# Autodesk Inventor assembly: Z Belt Drive Unit B
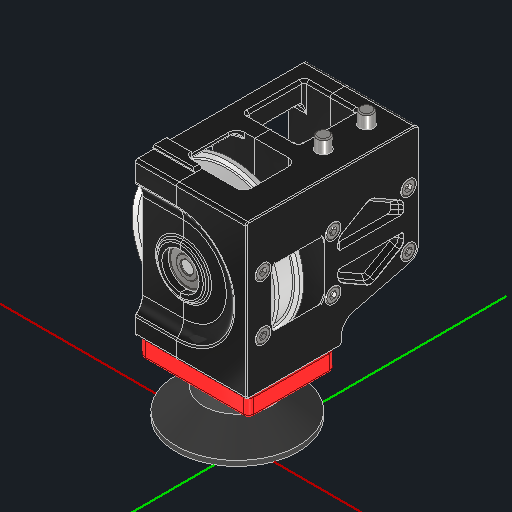
[picture p0: Inventor's stored thumbnail of the model, 512x512]
Saved by Autodesk Inventor 2022.2 (Build 262287010, 287A)
## iProperties
Created: 2022-03-12
Part Number: Z Belt Drive Unit B
Document SubType Name: Assembly
Designer: sleib
Author: sleib
## Documents named in this file (11)
- C:\Users\sleib\Projekte\Voron-2\CAD\Inventor\Z Belt-Drive Unit [B].iam
- C:\Users\sleib\Projekte\Voron-2\CAD\Inventor\Z Belt-Drive Body [B].ipt
- C:\Users\sleib\Projekte\Voron-2\CAD\Inventor\M3 Threaded Insert.ipt
- C:\Users\sleib\Projekte\Voron-2\CAD\Inventor\M3x40 SHCS.ipt
- C:\Users\sleib\Projekte\Voron-2\CAD\Inventor\M5x40 SHCS.ipt
- C:\Users\sleib\Projekte\Voron-2\CAD\Inventor\Z Belt-Drive Shaft.iam
- C:\Users\sleib\Projekte\Voron-2\CAD\Inventor\Z Belt-Drive Base-Plate [B].ipt
- C:\Users\sleib\Projekte\Voron-2\CAD\Inventor\M5x10 BHCS.ipt
- C:\Users\sleib\Projekte\Voron-2\CAD\Inventor\M5 Hexnut.ipt
- C:\Users\sleib\Projekte\Voron-2\CAD\Inventor\Rubber Compressor Foot.ipt
- C:\Users\sleib\Projekte\Voron-2\CAD\Inventor\M3x8 SHCS.ipt
## Components (26 placed, 10 different names)
1. Z Belt-Drive Body [B]:1 — Passend:1, Passend:2, Passend:3, Passend:4, Passend:5, Passend:6, Fluchtend:1, Fluchtend:2, Fluchtend:3, Fluchtend:4, Fluchtend:5, Fluchtend:6, Passend:7, Passend:8, Passend:9, Fluchtend:7, Fluchtend:8, Fluchtend:9, Passend:16, Passend:17, Passend:18, Passend:19, Passend:20, Passend:21, Passend:22, Passend:23, Passend:24, Passend:25, Passend:26, Passend:27, Passend:42, Passend:43, Fluchtend:45, Fluchtend:46
2. Z Belt-Drive Shaft:1 [sub-assembly] — Passend:26, Passend:27
3. Z Belt-Drive Base-Plate [B]:1 — Passend:28, Passend:29, Winkel:1, Passend:33, Passend:34, Passend:35, Passend:36, Passend:37, Passend:38, Passend:39, Passend:42
4. Rubber Compressor Foot:1 — Passend:30, Passend:31, Passend:33
5. M3 Threaded Insert:1 — Passend:1, Fluchtend:1, Passend:10
6. M3 Threaded Insert:2 — Passend:2, Fluchtend:2, Passend:11
7. M3 Threaded Insert:3 — Passend:3, Fluchtend:3, Passend:12
8. M3 Threaded Insert:4 — Passend:4, Fluchtend:4, Passend:13
9. M3 Threaded Insert:5 — Passend:5, Fluchtend:5, Passend:14
10. M3 Threaded Insert:6 — Passend:6, Fluchtend:6, Passend:15
11. M3 Threaded Insert:7 — Passend:7, Fluchtend:7, Passend:40
12. M3 Threaded Insert:8 — Passend:9, Fluchtend:9, Passend:41
13. M3 Threaded Insert:9 — Passend:8, Fluchtend:8
14. M3x40 SHCS:1 — Passend:10, Passend:16
15. M3x40 SHCS:2 — Passend:11, Passend:17
16. M3x40 SHCS:3 — Passend:12, Passend:18
17. M3x40 SHCS:4 — Passend:13, Passend:19
18. M3x40 SHCS:5 — Passend:14, Passend:20
19. M3x40 SHCS:6 — Passend:15, Passend:21
20. M5x40 SHCS:1 — Passend:22, Passend:24
21. M5x40 SHCS:2 — Passend:23, Passend:25
22. M5x10 BHCS:1 — Passend:30, Passend:31, Passend:32
23. M5 Hexnut:1 — Passend:28, Passend:29, Winkel:1, Passend:32
24. M3x8 SHCS:1 — Passend:34, Passend:37, Passend:40
25. M3x8 SHCS:2 — Passend:35, Passend:38
26. M3x8 SHCS:3 — Passend:36, Passend:39, Passend:41
## Relationships (55: Mate 43, Flush 11, Angle 1)
- Passend:1 [Mate]: Z Belt-Drive Body [B]:1 ↔ M3 Threaded Insert:1
- Passend:2 [Mate]: Z Belt-Drive Body [B]:1 ↔ M3 Threaded Insert:2
- Passend:3 [Mate]: Z Belt-Drive Body [B]:1 ↔ M3 Threaded Insert:3
- Passend:4 [Mate]: Z Belt-Drive Body [B]:1 ↔ M3 Threaded Insert:4
- Passend:5 [Mate]: Z Belt-Drive Body [B]:1 ↔ M3 Threaded Insert:5
- Passend:6 [Mate]: Z Belt-Drive Body [B]:1 ↔ M3 Threaded Insert:6
- Fluchtend:1 [Flush]: Z Belt-Drive Body [B]:1 ↔ M3 Threaded Insert:1
- Fluchtend:2 [Flush]: Z Belt-Drive Body [B]:1 ↔ M3 Threaded Insert:2
- Fluchtend:3 [Flush]: Z Belt-Drive Body [B]:1 ↔ M3 Threaded Insert:3
- Fluchtend:4 [Flush]: Z Belt-Drive Body [B]:1 ↔ M3 Threaded Insert:4
- Fluchtend:5 [Flush]: Z Belt-Drive Body [B]:1 ↔ M3 Threaded Insert:5
- Fluchtend:6 [Flush]: Z Belt-Drive Body [B]:1 ↔ M3 Threaded Insert:6
- Passend:7 [Mate]: Z Belt-Drive Body [B]:1 ↔ M3 Threaded Insert:7
- Passend:8 [Mate]: Z Belt-Drive Body [B]:1 ↔ M3 Threaded Insert:9
- Passend:9 [Mate]: Z Belt-Drive Body [B]:1 ↔ M3 Threaded Insert:8
- Fluchtend:7 [Flush]: Z Belt-Drive Body [B]:1 ↔ M3 Threaded Insert:7
- Fluchtend:8 [Flush]: Z Belt-Drive Body [B]:1 ↔ M3 Threaded Insert:9
- Fluchtend:9 [Flush]: Z Belt-Drive Body [B]:1 ↔ M3 Threaded Insert:8
- Passend:10 [Mate]: M3 Threaded Insert:1 ↔ M3x40 SHCS:1
- Passend:11 [Mate]: M3 Threaded Insert:2 ↔ M3x40 SHCS:2
- Passend:12 [Mate]: M3 Threaded Insert:3 ↔ M3x40 SHCS:3
- Passend:13 [Mate]: M3 Threaded Insert:4 ↔ M3x40 SHCS:4
- Passend:14 [Mate]: M3 Threaded Insert:5 ↔ M3x40 SHCS:5
- Passend:15 [Mate]: M3 Threaded Insert:6 ↔ M3x40 SHCS:6
- Passend:16 [Mate]: Z Belt-Drive Body [B]:1 ↔ M3x40 SHCS:1
- Passend:17 [Mate]: Z Belt-Drive Body [B]:1 ↔ M3x40 SHCS:2
- Passend:18 [Mate]: Z Belt-Drive Body [B]:1 ↔ M3x40 SHCS:3
- Passend:19 [Mate]: Z Belt-Drive Body [B]:1 ↔ M3x40 SHCS:4
- Passend:20 [Mate]: Z Belt-Drive Body [B]:1 ↔ M3x40 SHCS:5
- Passend:21 [Mate]: Z Belt-Drive Body [B]:1 ↔ M3x40 SHCS:6
- Passend:22 [Mate]: Z Belt-Drive Body [B]:1 ↔ M5x40 SHCS:1
- Passend:23 [Mate]: Z Belt-Drive Body [B]:1 ↔ M5x40 SHCS:2
- Passend:24 [Mate]: Z Belt-Drive Body [B]:1 ↔ M5x40 SHCS:1
- Passend:25 [Mate]: Z Belt-Drive Body [B]:1 ↔ M5x40 SHCS:2
- Passend:26 [Mate]: Z Belt-Drive Body [B]:1 ↔ Z Belt-Drive Shaft:1
- Passend:27 [Mate]: Z Belt-Drive Body [B]:1 ↔ Z Belt-Drive Shaft:1
- Passend:28 [Mate]: Z Belt-Drive Base-Plate [B]:1 ↔ M5 Hexnut:1
- Passend:29 [Mate]: Z Belt-Drive Base-Plate [B]:1 ↔ M5 Hexnut:1
- Winkel:1 [Angle] (0 deg): Z Belt-Drive Base-Plate [B]:1 ↔ M5 Hexnut:1
- Passend:30 [Mate]: Rubber Compressor Foot:1 ↔ M5x10 BHCS:1
- Passend:31 [Mate]: Rubber Compressor Foot:1 ↔ M5x10 BHCS:1
- Passend:32 [Mate]: M5x10 BHCS:1 ↔ M5 Hexnut:1
- Passend:33 [Mate]: Z Belt-Drive Base-Plate [B]:1 ↔ Rubber Compressor Foot:1
- Passend:34 [Mate]: Z Belt-Drive Base-Plate [B]:1 ↔ M3x8 SHCS:1
- Passend:35 [Mate]: Z Belt-Drive Base-Plate [B]:1 ↔ M3x8 SHCS:2
- Passend:36 [Mate]: Z Belt-Drive Base-Plate [B]:1 ↔ M3x8 SHCS:3
- Passend:37 [Mate]: Z Belt-Drive Base-Plate [B]:1 ↔ M3x8 SHCS:1
- Passend:38 [Mate]: Z Belt-Drive Base-Plate [B]:1 ↔ M3x8 SHCS:2
- Passend:39 [Mate]: Z Belt-Drive Base-Plate [B]:1 ↔ M3x8 SHCS:3
- Passend:40 [Mate]: M3 Threaded Insert:7 ↔ M3x8 SHCS:1
- Passend:41 [Mate]: M3 Threaded Insert:8 ↔ M3x8 SHCS:3
- Passend:42 [Mate]: Z Belt-Drive Body [B]:1 ↔ Z Belt-Drive Base-Plate [B]:1
- Passend:43 [Mate] (-10 mm): Z Belt-Drive Body [B]:1
- Fluchtend:45 [Flush] (-10 mm): Z Belt-Drive Body [B]:1
- Fluchtend:46 [Flush]: Z Belt-Drive Body [B]:1
